# Autodesk Inventor assembly: SP16-2P female waterproof connector
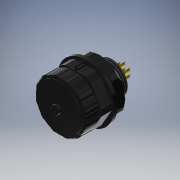
[picture p0: Inventor's stored thumbnail of the model, 180x180]
Saved by Autodesk Inventor 2018 (Build 220112000, 112)
## iProperties
Created: 2019-04-16
Part Number: SP16-2P female waterproof connector
Document SubType Name: Assembly
Designer: ZEUSLAP
Author: ZEUSLAP
## Documents named in this file (6)
- C:\Users\Vadim\Desktop\sp16-waterproof-connector-1.snapshot.3ffdsfds\SP16-7P, female, back nut type.iam
- C:\Users\Vadim\Desktop\sp16-waterproof-connector-1.snapshot.3ffdsfds\parts\cap.ipt
- C:\Users\Vadim\Desktop\sp16-waterproof-connector-1.snapshot.3ffdsfds\parts\rubber_washer.ipt
- C:\Users\Vadim\Desktop\sp16-waterproof-connector-1.snapshot.3ffdsfds\parts\body.ipt
- C:\Users\Vadim\Desktop\sp16-waterproof-connector-1.snapshot.3ffdsfds\parts\nut.ipt
- C:\Users\Vadim\Desktop\sp16-waterproof-connector-1.snapshot.3ffdsfds\parts\center_7p_female.iam
## Components (5 placed, 5 different names)
1. cap:1 — Mate:1, Mate:2, Mate:7
2. rubber_washer:1 — Mate:4, Mate:5, Mate:6
3. body:1 — Mate:1, Mate:2, Mate:3, Mate:4, Mate:5, Angle:1, Mate:8, Mate:9, Flush:1
4. nut:1 — Mate:3, Mate:6
5. center_7p_female:1 [sub-assembly] — Mate:8, Mate:9, Flush:1
## Relationships (11: Mate 9, Angle 1, Flush 1)
- Mate:1: cap:1 ↔ body:1
- Mate:2: cap:1 ↔ body:1
- Mate:3: body:1 ↔ nut:1
- Mate:4: rubber_washer:1 ↔ body:1
- Mate:5: rubber_washer:1 ↔ body:1
- Mate:6: rubber_washer:1 ↔ nut:1
- Mate:7: cap:1
- Angle:1 (180 deg): body:1
- Mate:8: body:1 ↔ center_7p_female:1
- Mate:9: body:1 ↔ center_7p_female:1
- Flush:1: body:1 ↔ center_7p_female:1
